# Autodesk Inventor assembly: ASY TRM 040 seal
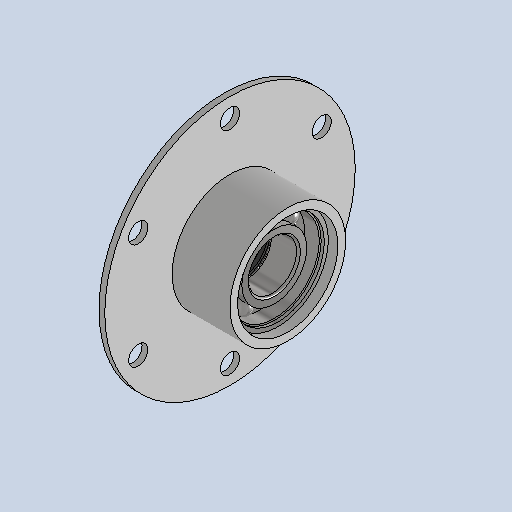
[picture p0: Inventor's stored thumbnail of the model, 512x512]
Saved by Autodesk Inventor 2025 (Build 290162010, 162A)
## iProperties
Created: 2024-09-08
Part Number: ASY TRM 040 seal
Document SubType Name: Assembly
Designer: pokla
Author: pokla
## Documents named in this file (6)
- C:\Users\admin\YandexDisk-badmisterfox\домашниий пк\Inventor\BSH_Beshkino_bio_tank\ASY TRM 040 seal.iam
- C:\Users\admin\YandexDisk-badmisterfox\домашниий пк\Inventor\BSH_Beshkino_bio_tank\TRM 041 flange.ipt
- C:\Users\admin\YandexDisk-badmisterfox\домашниий пк\Inventor\BSH_Beshkino_bio_tank\TRM 042 flange tube.ipt
- C:\Users\admin\YandexDisk-badmisterfox\домашниий пк\Inventor\BSH_Beshkino_bio_tank\ANSI B 27.7M - 3BMI-50.ipt
- C:\Users\admin\YandexDisk-badmisterfox\домашниий пк\Inventor\BSH_Beshkino_bio_tank\BS 290 SKF - SKF 7205 BE.ipt
- C:\Users\admin\YandexDisk-badmisterfox\домашниий пк\Inventor\BSH_Beshkino_bio_tank\CSN 02 9401 - G 25x52x7 - NBR.ipt
## Components (5 placed, 5 different names)
1. TRM 041 flange:1 — Rigid:2, Rigid:3
2. TRM 042 flange tube:1 — Rigid:4
3. ANSI B 27.7M 3BMI-50:1 — Rigid:4
4. BS 290 SKF SKF 7205 BE:1 — Rigid:3
5. CSN 02 9401 G G 25x52x7 - NBR:1 — Rigid:2
## Relationships (4: WeldJoint 4)
- [WeldJoint]: TRM 041 flange:1 ↔ TRM 042 flange tube:1
- Rigid:2 [WeldJoint]: TRM 041 flange:1 ↔ CSN 02 9401 G G 25x52x7 - NBR:1
- Rigid:3 [WeldJoint] (-8 mm): TRM 041 flange:1 ↔ BS 290 SKF SKF 7205 BE:1
- Rigid:4 [WeldJoint]: TRM 042 flange tube:1 ↔ ANSI B 27.7M 3BMI-50:1
